# Autodesk Inventor assembly: SINGLE_SYRINGE_ASSEMBLY
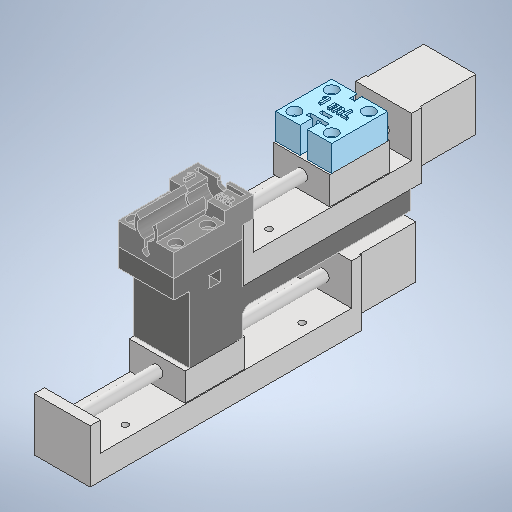
[picture p0: Inventor's stored thumbnail of the model, 512x512]
Saved by Autodesk Inventor 2025.2 (Build 292293000, 293)
## iProperties
Created: 2026-02-09
Part Number: SINGLE_SYRINGE_ASSEMBLY
Document SubType Name: Assembly
Designer: composite
Author: composite
## Documents named in this file (6)
- H:\01-Members Space\Sam Munro\Extrusion Printer\Printer V2\PRINTESS FILES\SINGLE_SYRINGE_ASSEMBLY.iam
- H:\01-Members Space\Sam Munro\Extrusion Printer\Printer V2\PRINTESS FILES\AE_100MM_ASSEM.iam
- H:\01-Members Space\Sam Munro\Extrusion Printer\Printer V2\PRINTESS FILES\Z-Axes Holder\Z-Axes Holder.ipt
- H:\01-Members Space\Sam Munro\Extrusion Printer\Printer V2\PRINTESS FILES\AE_50MM_ASSEM.iam
- H:\01-Members Space\Sam Munro\Extrusion Printer\Printer V2\PRINTESS FILES\1mL Plunger Holder\1mL Plunger Holder.ipt
- H:\01-Members Space\Sam Munro\Extrusion Printer\Printer V2\PRINTESS FILES\1mL Barrel Holder\1mL Barrel Holder.ipt
## Components (5 placed, 5 different names)
1. AE_100MM_ASSEM:1 [sub-assembly] — Mate:1, Mate:2, Mate:3
2. Z-Axes Holder:1 — Mate:1, Mate:2, Mate:3, Mate:4, Mate:5, Mate:6, Mate:10, Mate:11, Mate:12
3. AE_50MM_ASSEM:1 [sub-assembly] — Mate:4, Mate:5, Mate:6, Mate:7, Mate:8, Mate:9
4. 1mL Plunger Holder:1 — Mate:7, Mate:8, Mate:9
5. 1mL Barrel Holder:1 — Mate:10, Mate:11, Mate:12
## Relationships (12: Mate 12)
- Mate:1: AE_100MM_ASSEM:1 ↔ Z-Axes Holder:1
- Mate:2: AE_100MM_ASSEM:1 ↔ Z-Axes Holder:1
- Mate:3: AE_100MM_ASSEM:1 ↔ Z-Axes Holder:1
- Mate:4: Z-Axes Holder:1 ↔ AE_50MM_ASSEM:1
- Mate:5: Z-Axes Holder:1 ↔ AE_50MM_ASSEM:1
- Mate:6: Z-Axes Holder:1 ↔ AE_50MM_ASSEM:1
- Mate:7: AE_50MM_ASSEM:1 ↔ 1mL Plunger Holder:1
- Mate:8: AE_50MM_ASSEM:1 ↔ 1mL Plunger Holder:1
- Mate:9: AE_50MM_ASSEM:1 ↔ 1mL Plunger Holder:1
- Mate:10: Z-Axes Holder:1 ↔ 1mL Barrel Holder:1
- Mate:11: Z-Axes Holder:1 ↔ 1mL Barrel Holder:1
- Mate:12: Z-Axes Holder:1 ↔ 1mL Barrel Holder:1
